# Autodesk Inventor assembly: 000 - OmniBot
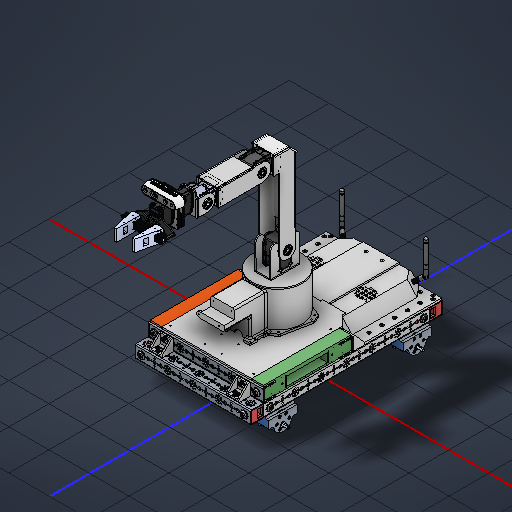
[picture p0: Inventor's stored thumbnail of the model, 512x512]
Saved by Autodesk Inventor 2025 (Build 290162000, 162)
## iProperties
Created: 2022-01-16
Part Number: 000 - OmniBot
Document SubType Name: Assembly
Designer: Петров Иван
Author: Петров Иван
## Documents named in this file (3)
- D:\Projects\OmniBot\design\000.000 - OmniBot.iam
- D:\Projects\OmniBot\design\000.001 - Ходовая часть.iam
- D:\Projects\OmniBot\design\Манипулятор AR\Угловой v5.iam
## Components (2 placed, 2 different names)
1. 000.001 - Ходовая часть:1 [sub-assembly] — Совмещение:1, Совмещение:2, Совмещение:3, Совмещение:4
2. Угловой v5:1 [sub-assembly] — Совмещение:1, Совмещение:2, Совмещение:3, Совмещение:4
## Relationships (4: Mate 4)
- Совмещение:1 [Mate]: 000.001 - Ходовая часть:1 ↔ Угловой v5:1
- Совмещение:2 [Mate]: 000.001 - Ходовая часть:1 ↔ Угловой v5:1
- Совмещение:3 [Mate]: 000.001 - Ходовая часть:1 ↔ Угловой v5:1
- Совмещение:4 [Mate]: 000.001 - Ходовая часть:1 ↔ Угловой v5:1
